# Autodesk Inventor assembly: TopIMU
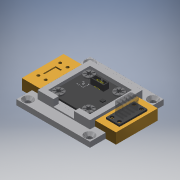
[picture p0: Inventor's stored thumbnail of the model, 180x180]
Saved by Autodesk Inventor 2019 (Build 230136000, 136)
## iProperties
Created: 2020-06-30
Part Number: TopIMU
Document SubType Name: Assembly
Designer: james
Author: james
## Documents named in this file (4)
- F:\JimsRobot\FIRSTRobots\Design\Library\Jims\TopIMU.iam
- F:\JimsRobot\FIRSTRobots\Design\Library\Jims\IMUWithCAN.iam
- F:\JimsRobot\FIRSTRobots\Design\Library\CTR\PIGEON_CAD\PIGEON_CAD\PIGEON.iam
- F:\JimsRobot\FIRSTRobots\Design\Library\CTR\CAN_CON_CAD\CAN_CON.ipt
## Components (3 placed, 3 different names)
1. IMUWithCAN:1 [sub-assembly] — Mate:1, Mate:2, Mate:3, Mate:4
2. PIGEON:1 [sub-assembly] — Mate:1, Mate:2
3. CAN_CON:1 — Mate:3, Mate:4
## Relationships (4: Mate 4)
- Mate:1 (3.81 mm): IMUWithCAN:1 ↔ PIGEON:1
- Mate:2: IMUWithCAN:1 ↔ PIGEON:1
- Mate:3: IMUWithCAN:1 ↔ CAN_CON:1
- Mate:4: IMUWithCAN:1 ↔ CAN_CON:1
